# Autodesk Inventor assembly: Better Syringe
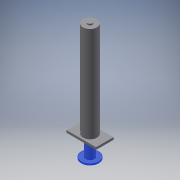
[picture p0: Inventor's stored thumbnail of the model, 180x180]
Saved by Autodesk Inventor 2019 (Build 230136000, 136)
## iProperties
Created: 2019-06-10
Part Number: Better Syringe
Document SubType Name: Assembly
Designer: Cole
Author: Cole
## Documents named in this file (3)
- G:\My Drive\Clubs\MTHS TSA\Animatronics 2019\Glyptodon\Glyptodon Work\MudBox Exports\Better Syringe.iam
- G:\My Drive\Clubs\MTHS TSA\Animatronics 2019\Glyptodon\Glyptodon Work\Syringe3mL\SyringeBody.ipt
- G:\My Drive\Clubs\MTHS TSA\Animatronics 2019\Glyptodon\Glyptodon Work\Syringe3mL\SyringEnd.ipt
## Components (2 placed, 2 different names)
1. SyringeBody:1 — Mate:1, Cylindrical:1
2. SyringEnd:1 — Mate:1, Cylindrical:1
## Relationships (2: Mate 1, CylindricalJoint 1)
- Mate:1: SyringeBody:1 ↔ SyringEnd:1
- Cylindrical:1: SyringeBody:1 ↔ SyringEnd:1
